# Autodesk Inventor assembly: CaseC
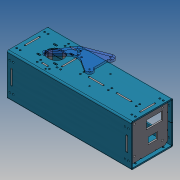
[picture p0: Inventor's stored thumbnail of the model, 180x180]
Saved by Autodesk Inventor 2017 (Build 210142000, 142)
## iProperties
Part Number: CaseC
Material: Genérico
Document SubType Name: Assembly
Designer: Leo
Author: Leo
## Documents named in this file (7)
- C:\Users\Leo\Dropbox\E\Caja Motriz\CaseC.iam
- C:\Users\Leo\Dropbox\E\Caja Motriz\Case\Protector.ipt
- C:\Users\Leo\Dropbox\E\Caja Motriz\Case\Refuerzo U.ipt
- C:\Users\Leo\Dropbox\E\Caja Motriz\Case\bandeja central.ipt
- C:\Users\Leo\Dropbox\E\Caja Motriz\Case\Tapa Enchufes.ipt
- C:\Users\Leo\Dropbox\E\Caja Motriz\Case\Pieza4.ipt
- C:\Users\Leo\Dropbox\E\Caja Motriz\Case\Pliegue Principal.ipt
## Components (6 placed, 6 different names)
1. Pliegue Principal:1 — Coincidencia:1, Nivelación:5, Nivelación:6, Nivelación:7, Coincidencia:2, Nivelación:8, Nivelación:10, Nivelación:11, Nivelación:13
2. Protector:1 — Nivelación:1, Nivelación:2, Nivelación:3
3. Refuerzo U:1 — Nivelación:4, Coincidencia:1, Nivelación:5
4. bandeja central:1 — Nivelación:6, Nivelación:7, Coincidencia:2
5. Tapa Enchufes:1 — Nivelación:8, Nivelación:9, Nivelación:10
6. Pieza4:1 — Nivelación:11, Nivelación:12, Nivelación:13
## Relationships (15: Flush 13, Mate 2)
- Nivelación:1 [Flush] (40 mm): Protector:1
- Nivelación:2 [Flush]: Protector:1
- Nivelación:3 [Flush]: Protector:1
- Nivelación:4 [Flush]: Refuerzo U:1
- Coincidencia:1 [Mate]: Pliegue Principal:1 ↔ Refuerzo U:1
- Nivelación:5 [Flush]: Pliegue Principal:1 ↔ Refuerzo U:1
- Nivelación:6 [Flush]: Pliegue Principal:1 ↔ bandeja central:1
- Nivelación:7 [Flush]: Pliegue Principal:1 ↔ bandeja central:1
- Coincidencia:2 [Mate]: Pliegue Principal:1 ↔ bandeja central:1
- Nivelación:8 [Flush]: Pliegue Principal:1 ↔ Tapa Enchufes:1
- Nivelación:9 [Flush]: Tapa Enchufes:1
- Nivelación:10 [Flush]: Pliegue Principal:1 ↔ Tapa Enchufes:1
- Nivelación:11 [Flush]: Pliegue Principal:1 ↔ Pieza4:1
- Nivelación:12 [Flush]: Pieza4:1
- Nivelación:13 [Flush]: Pliegue Principal:1 ↔ Pieza4:1
